# Autodesk Inventor assembly: bike_backup
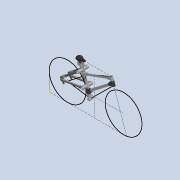
[picture p0: Inventor's stored thumbnail of the model, 180x180]
Saved by Autodesk Inventor 2021 (Build 250183000, 183)
## iProperties
RuleStatus: InUse
Created: 2020-04-29
Part Number: bike_backup
Document SubType Name: Assembly
Designer: Hannah
Mass: 8154.91 g
Surface Area: 13669.7 cm^2
Volume: 2710.91 cm^3
Density: 3.00818 g/cm^3
Author: Hannah
## Documents named in this file (20)
- \\Mac\Home\Documents\GitHub\AdjustaBike-2.0\CAD\bike_backup.iam
- \\Mac\Home\Documents\GitHub\AdjustaBike-2.0\CAD\prelim bike geo.ipt
- \\Mac\Home\Documents\GitHub\AdjustaBike-2.0\CAD\bottom bracket.ipt
- \\Mac\Home\Documents\GitHub\AdjustaBike-2.0\CAD\L10-7.ipt
- \\Mac\Home\Documents\GitHub\AdjustaBike-2.0\CAD\tube-08.ipt
- \\Mac\Home\Documents\GitHub\AdjustaBike-2.0\CAD\tube-09.ipt
- \\Mac\Home\Documents\GitHub\AdjustaBike-2.0\CAD\tube-10.ipt
- \\Mac\Home\Documents\GitHub\AdjustaBike-2.0\CAD\tube-12.ipt
- \\Mac\Home\Documents\GitHub\AdjustaBike-2.0\CAD\329-7.ipt
- \\Mac\Home\Documents\GitHub\AdjustaBike-2.0\CAD\head tube.ipt
- \\Mac\Home\Documents\GitHub\AdjustaBike-2.0\CAD\L26-7.ipt
- \\Mac\Home\Documents\GitHub\AdjustaBike-2.0\CAD\10-76.ipt
- \\Mac\Home\Documents\GitHub\AdjustaBike-2.0\CAD\LM51-6.ipt
- \\Mac\Home\Documents\GitHub\AdjustaBike-2.0\CAD\LF50-6.ipt
- \\Mac\Home\Documents\GitHub\AdjustaBike-2.0\CAD\tube-16.ipt
- \\Mac\Home\Documents\GitHub\AdjustaBike-2.0\CAD\tube-17.ipt
- \\Mac\Home\Documents\GitHub\AdjustaBike-2.0\CAD\saddle.ipt
- \\Mac\Home\Documents\GitHub\AdjustaBike-2.0\CAD\M51-5.ipt
- \\Mac\Home\Documents\GitHub\AdjustaBike-2.0\CAD\LM51-7.ipt
- \\Mac\Home\Documents\GitHub\AdjustaBike-2.0\CAD\link.ipt
## Components (36 placed, 19 different names)
1. prelim bike geo:1 — Mate:1, Mate:2, Angle:1, Mate:41
2. bottom bracket:1 — Mate:4, Flush:1, Mate:5, Mate:6, Tangent:1
3. L10-7:1 — Mate:6, Flush:2, Mate:7, Mate:9
4. seat tube — Mate:7, Tangent:1, Flush:9, Angle:2, Mate:8, Angle:5, Mate:17, Mate:19, Tangent:5, Tangent:6, Mate:24, Tangent:7, Tangent:8, Mate:28, Flush:21, Mate:96, Mate:99
5. down tube — Flush:10, Angle:3, Tangent:2, Mate:11, Tangent:3, Angle:4, Mate:12
6. top tube — Mate:16, Tangent:4, Mate:18
7. chainstay:1 — Mate:35, Tangent:11, Mate:39
8. chainstay:2 — Mate:36, Tangent:12, Mate:40
9. spacer:1 — Tangent:8, Flush:18, Mate:83, Mate:87, Tangent:13
10. spacer:2 — Tangent:7, Mate:30, Mate:34, Mate:84, Tangent:14
11. spacer:3 — Mate:23, Tangent:6, Angle:7, Mate:33, Flush:19, Tangent:12
12. spacer:4 — Mate:22, Tangent:5, Angle:6, Mate:32, Flush:17, Tangent:11
13. 329-7:1 — Mate:8, Mate:9, Mate:10, Angle:3, Tangent:2, Mate:11, Mate:21
14. 329-7:2 — Tangent:3, Angle:4, Mate:12, Mate:13, Mate:14, Flush:11
15. head tube:1 — Mate:14, Flush:11, Flush:12, Angle:5, Mate:15, Flush:13, Tangent:4
16. L10-7:2 — Mate:17, Mate:18, Mate:25
17. L10-7:3 — Mate:15, Flush:13, Flush:14, Mate:16
18. L26-7:1 — Mate:19, Mate:20, Mate:21, Mate:22, Mate:23
19. L26-7:2 — Mate:24, Flush:15, Mate:25, Mate:29, Mate:83, Mate:84
20. LM51-7:1 — Mate:28, Mate:29, Flush:16, Flush:21, Flush:22, Mate:98, Mate:100, Mate:101, Mate:102, Mate:103, Mate:106, Mate:108, Mate:109, Mate:110
21. 10-76:1 — Mate:33, Flush:19, Mate:36
22. 10-76:2 — Mate:32, Flush:17, Mate:35
23. 10-76:3 — Mate:30, Mate:34, Mate:89
24. 10-76:4 — Flush:18, Mate:87, Mate:88
25. LM51-6:1 — Mate:39, Angle:8, Mate:42, Mate:85, Mate:86, Mate:93, Mate:94
26. LM51-6:2 — Mate:40, Angle:9, Mate:43, Mate:85, Mate:92, Mate:95
27. LF50-6:2 — Angle:11, Mate:91, Mate:93, Mate:94
28. LF50-6:3 — Mate:90, Mate:92, Mate:95
29. tube-17:1 — Mate:88, Tangent:13, Mate:90
30. tube-17:2 — Mate:89, Tangent:14, Mate:91
31. saddle:1 — Mate:96, Flush:98, Mate:97
32. M51-5:1 — Mate:97, Mate:98, Mate:99, Mate:104, Mate:105, Mate:107, Mate:111
33. link:1 — Mate:100, Mate:106, Mate:111
34. link:2 — Mate:101, Mate:107, Mate:108
35. link:3 — Mate:102, Mate:104, Mate:110
36. link:4 — Mate:103, Mate:105, Mate:109
## Relationships (105: Mate 67, Flush 16, Tangent 12, Angle 10)
- Mate:1: prelim bike geo:1
- Mate:2: prelim bike geo:1
- Mate:3
- Mate:4: bottom bracket:1
- Flush:1: bottom bracket:1
- Angle:1 (0 deg): prelim bike geo:1
- Mate:5: bottom bracket:1
- Mate:6: bottom bracket:1 ↔ L10-7:1
- Flush:2: L10-7:1
- Mate:7: L10-7:1 ↔ seat tube
- Tangent:1: bottom bracket:1 ↔ seat tube
- Flush:9: seat tube
- Angle:2 (-70 deg): seat tube
- Flush:10: down tube
- Mate:8: seat tube ↔ 329-7:1
- Mate:9 (5 mm): L10-7:1 ↔ 329-7:1
- Mate:10: 329-7:1
- Angle:3 (72 deg): down tube ↔ 329-7:1
- Tangent:2: down tube ↔ 329-7:1
- Mate:11: down tube ↔ 329-7:1
- Tangent:3: down tube ↔ 329-7:2
- Angle:4 (0 deg): down tube ↔ 329-7:2
- Mate:12: down tube ↔ 329-7:2
- Mate:13: 329-7:2
- Mate:14: 329-7:2 ↔ head tube:1
- Flush:11: 329-7:2 ↔ head tube:1
- Flush:12: head tube:1
- Angle:5 (0 deg): seat tube ↔ head tube:1
- Mate:15: head tube:1 ↔ L10-7:3
- Flush:13: head tube:1 ↔ L10-7:3
- Flush:14: L10-7:3
- Mate:16: top tube ↔ L10-7:3
- Tangent:4: top tube ↔ head tube:1
- Mate:17: seat tube ↔ L10-7:2
- Mate:18: top tube ↔ L10-7:2
- Mate:19: seat tube ↔ L26-7:1
- Mate:20: L26-7:1
- Mate:21 (5 mm): 329-7:1 ↔ L26-7:1
- Mate:22: spacer:4 ↔ L26-7:1
- Tangent:5: seat tube ↔ spacer:4
- Angle:6 (0 deg): spacer:4
- Mate:23: spacer:3 ↔ L26-7:1
- Tangent:6: seat tube ↔ spacer:3
- Angle:7 (0 deg): spacer:3
- Mate:24: seat tube ↔ L26-7:2
- Flush:15: L26-7:2
- Mate:25 (5 mm): L10-7:2 ↔ L26-7:2
- Tangent:7: seat tube ↔ spacer:2
- Tangent:8: seat tube ↔ spacer:1
- Mate:28: seat tube ↔ LM51-7:1
- Mate:29 (5 mm): L26-7:2 ↔ LM51-7:1
- Flush:16: LM51-7:1
- Mate:30: spacer:2 ↔ 10-76:3
- Mate:32: spacer:4 ↔ 10-76:2
- Mate:33: spacer:3 ↔ 10-76:1
- Mate:34: spacer:2 ↔ 10-76:3
- Flush:17: spacer:4 ↔ 10-76:2
- Flush:18: spacer:1 ↔ 10-76:4
- Flush:19: spacer:3 ↔ 10-76:1
- Mate:35: chainstay:1 ↔ 10-76:2
- Mate:36: chainstay:2 ↔ 10-76:1
- Tangent:11: chainstay:1 ↔ spacer:4
- Tangent:12: chainstay:2 ↔ spacer:3
- Mate:39: chainstay:1 ↔ LM51-6:1
- Mate:40: chainstay:2 ↔ LM51-6:2
- Angle:8 (0 deg): LM51-6:1
- Angle:9 (0 deg): LM51-6:2
- Mate:41: prelim bike geo:1
- Mate:42: LM51-6:1
- Mate:43: LM51-6:2
- Angle:11 (0 deg): LF50-6:2
- Flush:21: seat tube ↔ LM51-7:1
- Flush:22: LM51-7:1
- Mate:83: spacer:1 ↔ L26-7:2
- Mate:84: spacer:2 ↔ L26-7:2
- Mate:85: LM51-6:1 ↔ LM51-6:2
- Mate:86: LM51-6:1
- Mate:87: spacer:1 ↔ 10-76:4
- Mate:88: 10-76:4 ↔ tube-17:1
- Mate:89: 10-76:3 ↔ tube-17:2
- Tangent:13: spacer:1 ↔ tube-17:1
- Tangent:14: spacer:2 ↔ tube-17:2
- Mate:90: LF50-6:3 ↔ tube-17:1
- Mate:91: LF50-6:2 ↔ tube-17:2
- Mate:92: LM51-6:2 ↔ LF50-6:3
- Mate:93: LM51-6:1 ↔ LF50-6:2
- Mate:94: LM51-6:1 ↔ LF50-6:2
- Mate:95: LM51-6:2 ↔ LF50-6:3
- Mate:96: seat tube ↔ saddle:1
- Flush:98: saddle:1
- Mate:97: saddle:1 ↔ M51-5:1
- Mate:98: LM51-7:1 ↔ M51-5:1
- Mate:99: seat tube ↔ M51-5:1
- Mate:100: LM51-7:1 ↔ link:1
- Mate:101: LM51-7:1 ↔ link:2
- Mate:102: LM51-7:1 ↔ link:3
- Mate:103: LM51-7:1 ↔ link:4
- Mate:104: M51-5:1 ↔ link:3
- Mate:105: M51-5:1 ↔ link:4
- Mate:106: LM51-7:1 ↔ link:1
- Mate:107: M51-5:1 ↔ link:2
- Mate:108: LM51-7:1 ↔ link:2
- Mate:109: LM51-7:1 ↔ link:4
- Mate:110: LM51-7:1 ↔ link:3
- Mate:111: M51-5:1 ↔ link:1
## Named parameters: Lst = 500 mm, Sst = 7, Ldt = 500 mm, Sdt = 7, Ltt = 516 mm, Stt = 7, Lcs = 330 mm, Scs = 6, Lss = 330 mm, Sss = 6, Lsp = 90 mm, Ssp = 7, Lcsn = 230 mm, Scsn = 7
